# Autodesk Inventor assembly: 1120_Shift Coil Assembly_V1
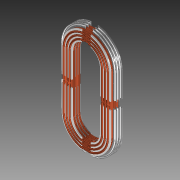
[picture p0: Inventor's stored thumbnail of the model, 180x180]
Saved by Autodesk Inventor 2020 (Build 240168000, 168)
## iProperties
Created: 2019-10-13
Part Number: 1120_Shift Coil Assembly_V1
Document SubType Name: Assembly
Designer: RFLab
Author: RFLab
## Documents named in this file (6)
- C:\Users\RFLab\Dropbox\MPI Group Folder\fMPI (Rodent)\Small Bore Imager_Open Source Files\Inventor Files\1xxx_Rotating Gantry\11xx_Magnet Assembly\1120_Shift Coil Assembly_V1.iam
- C:\Users\RFLab\Dropbox\MPI Group Folder\fMPI (Rodent)\Small Bore Imager_Open Source Files\Inventor Files\1xxx_Rotating Gantry\11xx_Magnet Assembly\112x_Shift Coil Assembly\1121_Shift Coils SubAssembly_V1.iam
- C:\Users\RFLab\Dropbox\MPI Group Folder\fMPI (Rodent)\Small Bore Imager_Open Source Files\Inventor Files\1xxx_Rotating Gantry\11xx_Magnet Assembly\112x_Shift Coil Assembly\1122_Middle Heat Sink_V1.ipt
- C:\Users\RFLab\Dropbox\MPI Group Folder\fMPI (Rodent)\Small Bore Imager_Open Source Files\Inventor Files\1xxx_Rotating Gantry\11xx_Magnet Assembly\112x_Shift Coil Assembly\1122A_Middle Heat Sink Mirror_V1.ipt
- C:\Users\RFLab\Dropbox\MPI Group Folder\fMPI (Rodent)\Small Bore Imager_Open Source Files\Inventor Files\1xxx_Rotating Gantry\11xx_Magnet Assembly\112x_Shift Coil Assembly\1123_Top Heat Sink_V1.ipt
- C:\Users\RFLab\Dropbox\MPI Group Folder\fMPI (Rodent)\Small Bore Imager_Open Source Files\Inventor Files\1xxx_Rotating Gantry\11xx_Magnet Assembly\112x_Shift Coil Assembly\1123B_Top Heat Sink Mirror_V1.ipt
## Components (19 placed, 5 different names)
1. 1121_Shift Coils SubAssembly_V1:1 [sub-assembly] — Mate:1, Mate:2, Flush:1, Mate:3, Mate:4, Angle:1, Mate:5, Flush:27
2. 1122_Middle Heat Sink_V1:1 — Mate:3, Mate:4, Angle:1, Flush:2, Angle:2, Flush:5, Flush:8, Mate:11
3. 1122_Middle Heat Sink_V1:2 — Flush:2, Mate:5, Angle:2, Flush:3, Flush:6, Flush:7, Mate:9, Tangent:1, Mate:12
4. 1122A_Middle Heat Sink Mirror_V1:1 — Flush:3, Flush:4, Flush:5, Flush:7
5. 1122A_Middle Heat Sink Mirror_V1:2 — Flush:4, Flush:6, Flush:8, Mate:10, Tangent:2, Flush:28
6. 1121_Shift Coils SubAssembly_V1:2 [sub-assembly] — Tangent:1, Tangent:2
7. 1122_Middle Heat Sink_V1:3 — Flush:28, Mate:15
8. 1122_Middle Heat Sink_V1:4 — Mate:12, Tangent:4, Mate:13, Mate:16
9. 1122A_Middle Heat Sink Mirror_V1:3 — Mate:14
10. 1122A_Middle Heat Sink Mirror_V1:4 — Tangent:3, Flush:36
11. 1122_Middle Heat Sink_V1:5 — Flush:24, Flush:25, Flush:26, Mate:11
12. 1122_Middle Heat Sink_V1:6 — Flush:23, Flush:27, Mate:9
13. 1122A_Middle Heat Sink Mirror_V1:5 — Flush:25
14. 1122A_Middle Heat Sink Mirror_V1:6 — Flush:23, Flush:24, Flush:26, Mate:10
15. 1121_Shift Coils SubAssembly_V1:3 [sub-assembly] — Tangent:3, Tangent:4, Mate:13, Mate:14, Tangent:5
16. 1123_Top Heat Sink_V1:1 — Flush:30, Flush:31, Flush:33, Flush:35, Mate:16
17. 1123_Top Heat Sink_V1:2 — Flush:29, Flush:30, Flush:32, Flush:34
18. 1123B_Top Heat Sink Mirror_V1:1 — Flush:31, Flush:33, Flush:34, Tangent:5, Mate:15
19. 1123B_Top Heat Sink Mirror_V1:2 — Flush:29, Flush:32, Flush:35, Flush:36
## Relationships (62: Flush 36, Mate 16, Angle 5, Tangent 5)
- Mate:1: 1121_Shift Coils SubAssembly_V1:1
- Mate:2: 1121_Shift Coils SubAssembly_V1:1
- Flush:1: 1121_Shift Coils SubAssembly_V1:1
- Mate:3: 1121_Shift Coils SubAssembly_V1:1 ↔ 1122_Middle Heat Sink_V1:1
- Mate:4: 1121_Shift Coils SubAssembly_V1:1 ↔ 1122_Middle Heat Sink_V1:1
- Angle:1 (180 deg): 1121_Shift Coils SubAssembly_V1:1 ↔ 1122_Middle Heat Sink_V1:1
- Flush:2: 1122_Middle Heat Sink_V1:1 ↔ 1122_Middle Heat Sink_V1:2
- Mate:5: 1121_Shift Coils SubAssembly_V1:1 ↔ 1122_Middle Heat Sink_V1:2
- Angle:2 (180 deg): 1122_Middle Heat Sink_V1:1 ↔ 1122_Middle Heat Sink_V1:2
- Flush:3: 1122_Middle Heat Sink_V1:2 ↔ 1122A_Middle Heat Sink Mirror_V1:1
- Flush:4: 1122A_Middle Heat Sink Mirror_V1:1 ↔ 1122A_Middle Heat Sink Mirror_V1:2
- Flush:5: 1122_Middle Heat Sink_V1:1 ↔ 1122A_Middle Heat Sink Mirror_V1:1
- Flush:6: 1122_Middle Heat Sink_V1:2 ↔ 1122A_Middle Heat Sink Mirror_V1:2
- Flush:7: 1122_Middle Heat Sink_V1:2 ↔ 1122A_Middle Heat Sink Mirror_V1:1
- Flush:8: 1122_Middle Heat Sink_V1:1 ↔ 1122A_Middle Heat Sink Mirror_V1:2
- [Mate]: 1121_Shift Coils SubAssembly_V1:2 ↔ 1122_Middle Heat Sink_V1:3
- [Mate]: 1121_Shift Coils SubAssembly_V1:2 ↔ 1122_Middle Heat Sink_V1:3
- [Angle] (180 deg): 1121_Shift Coils SubAssembly_V1:2 ↔ 1122_Middle Heat Sink_V1:3
- [Flush]: 1122_Middle Heat Sink_V1:3 ↔ 1122_Middle Heat Sink_V1:4
- [Mate]: 1121_Shift Coils SubAssembly_V1:2 ↔ 1122_Middle Heat Sink_V1:4
- [Angle] (180 deg): 1122_Middle Heat Sink_V1:3 ↔ 1122_Middle Heat Sink_V1:4
- [Flush]: 1122_Middle Heat Sink_V1:4 ↔ 1122A_Middle Heat Sink Mirror_V1:3
- [Flush]: 1122A_Middle Heat Sink Mirror_V1:3 ↔ 1122A_Middle Heat Sink Mirror_V1:4
- [Flush]: 1122_Middle Heat Sink_V1:3 ↔ 1122A_Middle Heat Sink Mirror_V1:3
- [Flush]: 1122_Middle Heat Sink_V1:4 ↔ 1122A_Middle Heat Sink Mirror_V1:4
- [Flush]: 1122_Middle Heat Sink_V1:4 ↔ 1122A_Middle Heat Sink Mirror_V1:3
- [Flush]: 1122_Middle Heat Sink_V1:3 ↔ 1122A_Middle Heat Sink Mirror_V1:4
- [Flush]: 1122_Middle Heat Sink_V1:5 ↔ 1122_Middle Heat Sink_V1:6
- [Angle] (180 deg): 1122_Middle Heat Sink_V1:5 ↔ 1122_Middle Heat Sink_V1:6
- [Flush]: 1122_Middle Heat Sink_V1:6 ↔ 1122A_Middle Heat Sink Mirror_V1:5
- [Flush]: 1122A_Middle Heat Sink Mirror_V1:5 ↔ 1122A_Middle Heat Sink Mirror_V1:6
- [Flush]: 1122_Middle Heat Sink_V1:5 ↔ 1122A_Middle Heat Sink Mirror_V1:5
- [Flush]: 1122_Middle Heat Sink_V1:6 ↔ 1122A_Middle Heat Sink Mirror_V1:6
- [Flush]: 1122_Middle Heat Sink_V1:6 ↔ 1122A_Middle Heat Sink Mirror_V1:5
- [Flush]: 1122_Middle Heat Sink_V1:5 ↔ 1122A_Middle Heat Sink Mirror_V1:6
- Flush:23: 1122_Middle Heat Sink_V1:6 ↔ 1122A_Middle Heat Sink Mirror_V1:6
- Flush:24: 1122_Middle Heat Sink_V1:5 ↔ 1122A_Middle Heat Sink Mirror_V1:6
- Flush:25: 1122_Middle Heat Sink_V1:5 ↔ 1122A_Middle Heat Sink Mirror_V1:5
- Flush:26: 1122_Middle Heat Sink_V1:5 ↔ 1122A_Middle Heat Sink Mirror_V1:6
- Flush:27: 1121_Shift Coils SubAssembly_V1:1 ↔ 1122_Middle Heat Sink_V1:6
- Mate:9: 1122_Middle Heat Sink_V1:2 ↔ 1122_Middle Heat Sink_V1:6
- Mate:10: 1122A_Middle Heat Sink Mirror_V1:2 ↔ 1122A_Middle Heat Sink Mirror_V1:6
- Mate:11: 1122_Middle Heat Sink_V1:1 ↔ 1122_Middle Heat Sink_V1:5
- Tangent:1: 1122_Middle Heat Sink_V1:2 ↔ 1121_Shift Coils SubAssembly_V1:2
- Tangent:2: 1122A_Middle Heat Sink Mirror_V1:2 ↔ 1121_Shift Coils SubAssembly_V1:2
- Flush:28: 1122A_Middle Heat Sink Mirror_V1:2 ↔ 1122_Middle Heat Sink_V1:3
- Mate:12: 1122_Middle Heat Sink_V1:2 ↔ 1122_Middle Heat Sink_V1:4
- Tangent:3: 1122A_Middle Heat Sink Mirror_V1:4 ↔ 1121_Shift Coils SubAssembly_V1:3
- Tangent:4: 1122_Middle Heat Sink_V1:4 ↔ 1121_Shift Coils SubAssembly_V1:3
- Mate:13: 1122_Middle Heat Sink_V1:4 ↔ 1121_Shift Coils SubAssembly_V1:3
- Mate:14: 1122A_Middle Heat Sink Mirror_V1:3 ↔ 1121_Shift Coils SubAssembly_V1:3
- Flush:29: 1123_Top Heat Sink_V1:2 ↔ 1123B_Top Heat Sink Mirror_V1:2
- Flush:30: 1123_Top Heat Sink_V1:1 ↔ 1123_Top Heat Sink_V1:2
- Flush:31: 1123_Top Heat Sink_V1:1 ↔ 1123B_Top Heat Sink Mirror_V1:1
- Flush:32: 1123_Top Heat Sink_V1:2 ↔ 1123B_Top Heat Sink Mirror_V1:2
- Flush:33: 1123_Top Heat Sink_V1:1 ↔ 1123B_Top Heat Sink Mirror_V1:1
- Flush:34: 1123_Top Heat Sink_V1:2 ↔ 1123B_Top Heat Sink Mirror_V1:1
- Flush:35: 1123_Top Heat Sink_V1:1 ↔ 1123B_Top Heat Sink Mirror_V1:2
- Tangent:5: 1121_Shift Coils SubAssembly_V1:3 ↔ 1123B_Top Heat Sink Mirror_V1:1
- Mate:15: 1122_Middle Heat Sink_V1:3 ↔ 1123B_Top Heat Sink Mirror_V1:1
- Mate:16: 1122_Middle Heat Sink_V1:4 ↔ 1123_Top Heat Sink_V1:1
- Flush:36: 1122A_Middle Heat Sink Mirror_V1:4 ↔ 1123B_Top Heat Sink Mirror_V1:2
## Named parameters: d15_d3 = 0 mm, d16_d4 = 0 mm, d17_d5 = 180 deg, d18_d6 = 0 mm, d19_d7 = 0 mm, d20_d8 = 180 deg, d21_d9 = 0 mm, d22_d10 = 0 mm, d23_d11 = 0 mm, d24_d12 = 0 mm, d25_d13 = 0 mm, d26_d14 = 0 mm, d27_d6 = 0 mm, d28_d8 = 180 deg, d29_d9 = 0 mm, d30_d10 = 0 mm, d31_d11 = 0 mm, d32_d12 = 0 mm, d33_d13 = 0 mm, d34_d14 = 0 mm
